# Autodesk Inventor assembly: акб+фанера
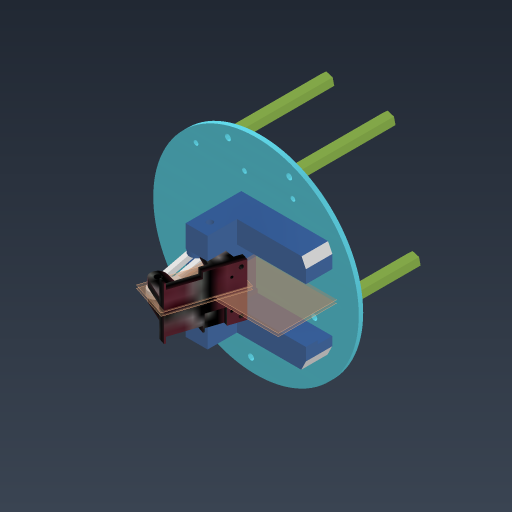
[picture p0: Inventor's stored thumbnail of the model, 512x512]
Saved by Autodesk Inventor 2023.2 (Build 272271030, 271C)
## iProperties
Created: 2024-03-01
Part Number: акб+фанера
Document SubType Name: Assembly
Designer: liza
Author: liza
## Documents named in this file (8)
- D:\!project\fox_n_crow_construction\crow\trunk\акб+фанера.iam
- D:\!project\fox_n_crow_construction\crow\trunk\фанера для акб.ipt
- C:\Users\liza\Desktop\Work\openmv3_export\KRAVT_holder_2.ipt
- D:\!project\fox_n_crow_construction\crow\trunk\стойка.ipt
- D:\!project\fox_n_crow_construction\crow\trunk\камера+качалка.iam
- D:\!project\fox_n_crow_construction\crow\trunk\кроншейн.ipt
- C:\Users\liza\Desktop\Work\openmv3_export\м4.ipt
- D:\!project\fox_n_crow_construction\crow\trunk\фанерная качалка.ipt
## Components (10 placed, 7 different names)
1. KRAVT_holder_2:1 — Совмещение:5
2. фанера для акб:1 — Совмещение:1, Совмещение:2, Совмещение:3, Совмещение:4, Совмещение:5, Вставка:1, Вставка:3, Заподлицо:2
3. стойка:1 — Совмещение:2, Вставка:1
4. стойка:2 — Совмещение:3, Вставка:3
5. стойка:3 — Совмещение:4
6. стойка:4 — Совмещение:1
7. камера+качалка:1 [sub-assembly] — Совмещение:6, Заподлицо:2, Совмещение:9, Цилиндрический:4
8. м4:1 — Заподлицо:1, Цилиндрический:3, Совмещение:9
9. кроншейн:1 — Совмещение:6, Заподлицо:1, Цилиндрический:3, Касательность:1, Совмещение:10
10. фанерная качалка:1 — Цилиндрический:4, Касательность:1, Совмещение:10
## Relationships (15: Mate 8, Insert 2, Flush 2, CylindricalJoint 2, Tangent 1)
- Совмещение:1 [Mate]: фанера для акб:1 ↔ стойка:4
- Совмещение:2 [Mate]: фанера для акб:1 ↔ стойка:1
- Совмещение:3 [Mate]: фанера для акб:1 ↔ стойка:2
- Совмещение:4 [Mate]: фанера для акб:1 ↔ стойка:3
- Совмещение:5 [Mate]: KRAVT_holder_2:1 ↔ фанера для акб:1
- Вставка:1 [Insert]: фанера для акб:1 ↔ стойка:1
- Вставка:3 [Insert]: фанера для акб:1 ↔ стойка:2
- Совмещение:6 [Mate] (0.5 mm): камера+качалка:1 ↔ кроншейн:1
- Заподлицо:1 [Flush] (16 mm): м4:1 ↔ кроншейн:1
- Заподлицо:2 [Flush]: фанера для акб:1 ↔ камера+качалка:1
- Цилиндрический:3 [CylindricalJoint]: м4:1 ↔ кроншейн:1
- Совмещение:9 [Mate]: камера+качалка:1 ↔ м4:1
- Цилиндрический:4 [CylindricalJoint]: камера+качалка:1 ↔ фанерная качалка:1
- Касательность:1 [Tangent]: кроншейн:1 ↔ фанерная качалка:1
- Совмещение:10 [Mate]: кроншейн:1 ↔ фанерная качалка:1
